# Autodesk Inventor assembly: Mx64_withHorn_andSchwung
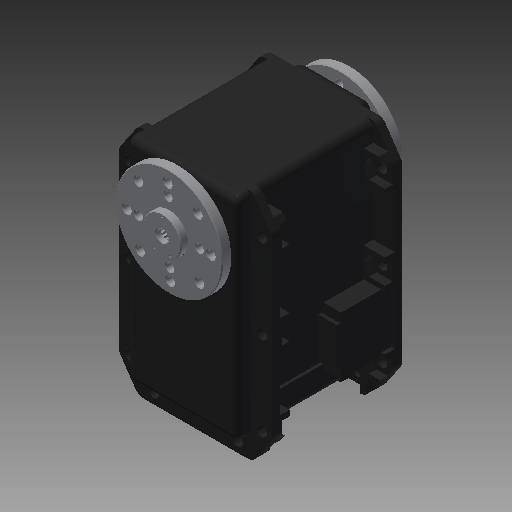
[picture p0: Inventor's stored thumbnail of the model, 512x512]
Saved by Autodesk Inventor 2018 (Build 220112000, 112)
## iProperties
Created: 2014-04-23
Part Number: Mx64_withHorn_andSchwung
Document SubType Name: Assembly
Designer: BitBots
Author: BitBots
## Documents named in this file (4)
- C:\Users\jaspe\bitbots_hardware\wolfgang\assembly\motors\MX64\Mx64_with_bearing.iam
- C:\Users\jaspe\bitbots_hardware\wolfgang\assembly\motors\MX64\MX64_body_modified.ipt
- C:\Users\jaspe\bitbots_hardware\wolfgang\assembly\motors\MX64\HN05-i1.ipt
- C:\Users\jaspe\bitbots_hardware\wolfgang\assembly\motors\MX64\HN05-N101.ipt
## Components (3 placed, 3 different names)
1. MX64_body_modified:1 — Rotational:4, Flush:1, Flush:2, Mate:1, Rotational:5
2. HN05-i1:1 — Rotational:4
3. HN05-N101:1 — Rotational:5
## Relationships (5: RevoluteJoint 2, Flush 2, Mate 1)
- Rotational:4 [RevoluteJoint]: MX64_body_modified:1 ↔ HN05-i1:1
- Flush:1: MX64_body_modified:1
- Flush:2: MX64_body_modified:1
- Mate:1: MX64_body_modified:1
- Rotational:5 [RevoluteJoint]: MX64_body_modified:1 ↔ HN05-N101:1
